# Autodesk Inventor assembly: DTFinal
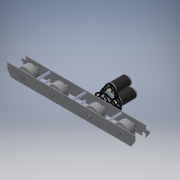
[picture p0: Inventor's stored thumbnail of the model, 180x180]
Saved by Autodesk Inventor 2016 (Build 200138000, 138)
## iProperties
Created: 2017-01-13
Part Number: DTFinal
Document SubType Name: Assembly
Designer: Kyle
Author: Kyle
## Documents named in this file (12)
- F:\FRC\2017\DriveTrain\DTFinal.iam
- F:\FRC\2017\DriveTrain\OutsidePlate.ipt
- F:\FRC\2017\DriveTrain\3.75Churro.ipt
- F:\FRC\2017\DriveTrain\8WDSingleSprocket.iam
- F:\FRC\2017\DriveTrain\8WDDoubleSprocket.iam
- F:\FRC\2017\DriveTrain\InsidePlate.ipt
- F:\FRC\2017\DriveTrain\WCPSS.iam
- F:\FRC\2017\DriveTrain\Individual parts\.5HexBearing.ipt
- F:\FRC\2017\DriveTrain\Individual parts\.5ShaftCollar.ipt
- F:\FRC\2017\DriveTrain\Individual parts\4x2Colson.ipt
- F:\FRC\2017\DriveTrain\Individual parts\16t25Sprocket.ipt
- F:\FRC\2017\DriveTrain\Individual parts\.144Spacer.ipt
## Components (20 placed, 11 different names)
1. OutsidePlate:1 — Mate:1, Mate:2, Mate:3, Mate:4, Mate:5, Mate:6, Mate:7, Mate:8, Mate:9, Mate:10, Mate:11, Mate:12, Mate:13, Mate:14, Mate:15, Mate:16, Mate:17, Mate:18, Mate:22, Mate:25
2. 3.75Churro:1 — Mate:2, Mate:18, Mate:19
3. 3.75Churro:2 — Mate:1, Mate:17
4. 3.75Churro:3 — Mate:4, Mate:16
5. 3.75Churro:4 — Mate:3, Mate:15
6. 3.75Churro:5 — Mate:6, Mate:14
7. 3.75Churro:6 — Mate:5, Mate:13, Mate:20, Mate:21
8. 8WDSingleSprocket:1 [sub-assembly] — Mate:9, Mate:10
9. 8WDSingleSprocket:2 [sub-assembly] — Mate:7, Mate:8
10. 8WDDoubleSprocket:1 [sub-assembly] — Mate:11, Mate:12
11. InsidePlate:1 — Mate:19, Mate:20, Mate:21, Mate:23, Mate:24, Mate:27
12. WCPSS:1 [sub-assembly] — Mate:26, Flush:1, Mate:27, Mate:28, Mate:30, Mate:32, Mate:34, Mate:36, Mate:38
13. .5HexBearing:1 — Mate:23, Mate:24, Mate:26, Mate:31
14. .5HexBearing:2 — Mate:22, Mate:25, Flush:1, Mate:29
15. .5ShaftCollar:1 — Mate:28, Mate:29, Mate:33
16. .5ShaftCollar:2 — Mate:30, Mate:31
17. 4x2Colson:1 — Mate:32, Mate:33, Mate:35
18. 16t25Sprocket:1 — Mate:34, Mate:35, Mate:37
19. 16t25Sprocket:2 — Mate:36, Mate:37, Mate:39
20. .144Spacer:1 — Mate:38, Mate:39
## Relationships (40: Mate 39, Flush 1)
- Mate:1: OutsidePlate:1 ↔ 3.75Churro:2
- Mate:2: OutsidePlate:1 ↔ 3.75Churro:1
- Mate:3: OutsidePlate:1 ↔ 3.75Churro:4
- Mate:4: OutsidePlate:1 ↔ 3.75Churro:3
- Mate:5: OutsidePlate:1 ↔ 3.75Churro:6
- Mate:6: OutsidePlate:1 ↔ 3.75Churro:5
- Mate:7: OutsidePlate:1 ↔ 8WDSingleSprocket:2
- Mate:8: OutsidePlate:1 ↔ 8WDSingleSprocket:2
- Mate:9: OutsidePlate:1 ↔ 8WDSingleSprocket:1
- Mate:10: OutsidePlate:1 ↔ 8WDSingleSprocket:1
- Mate:11: OutsidePlate:1 ↔ 8WDDoubleSprocket:1
- Mate:12: OutsidePlate:1 ↔ 8WDDoubleSprocket:1
- Mate:13: OutsidePlate:1 ↔ 3.75Churro:6
- Mate:14: OutsidePlate:1 ↔ 3.75Churro:5
- Mate:15: OutsidePlate:1 ↔ 3.75Churro:4
- Mate:16: OutsidePlate:1 ↔ 3.75Churro:3
- Mate:17: OutsidePlate:1 ↔ 3.75Churro:2
- Mate:18: OutsidePlate:1 ↔ 3.75Churro:1
- Mate:19: 3.75Churro:1 ↔ InsidePlate:1
- Mate:20: 3.75Churro:6 ↔ InsidePlate:1
- Mate:21: 3.75Churro:6 ↔ InsidePlate:1
- Mate:22: OutsidePlate:1 ↔ .5HexBearing:2
- Mate:23: InsidePlate:1 ↔ .5HexBearing:1
- Mate:24: InsidePlate:1 ↔ .5HexBearing:1
- Mate:25: OutsidePlate:1 ↔ .5HexBearing:2
- Mate:26: WCPSS:1 ↔ .5HexBearing:1
- Flush:1: WCPSS:1 ↔ .5HexBearing:2
- Mate:27: InsidePlate:1 ↔ WCPSS:1
- Mate:28: WCPSS:1 ↔ .5ShaftCollar:1
- Mate:29: .5HexBearing:2 ↔ .5ShaftCollar:1
- Mate:30: WCPSS:1 ↔ .5ShaftCollar:2
- Mate:31: .5HexBearing:1 ↔ .5ShaftCollar:2
- Mate:32: WCPSS:1 ↔ 4x2Colson:1
- Mate:33: .5ShaftCollar:1 ↔ 4x2Colson:1
- Mate:34: WCPSS:1 ↔ 16t25Sprocket:1
- Mate:35: 4x2Colson:1 ↔ 16t25Sprocket:1
- Mate:36: WCPSS:1 ↔ 16t25Sprocket:2
- Mate:37: 16t25Sprocket:1 ↔ 16t25Sprocket:2
- Mate:38: WCPSS:1 ↔ .144Spacer:1
- Mate:39: 16t25Sprocket:2 ↔ .144Spacer:1
